# Autodesk Inventor assembly: Placa_base
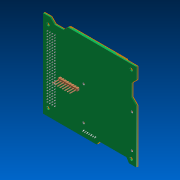
[picture p0: Inventor's stored thumbnail of the model, 180x180]
Saved by Autodesk Inventor 2012 (Build 160160000, 160)
## iProperties
Created: 2015-11-18
Part Number: Placa_base
Document SubType Name: Assembly
Designer: Alex Becerra
Mass: 39.7059 g
Surface Area: 235.798 cm^2
Volume: 15.4172 cm^3
Density: 2.57542 g/cm^3
Author: Alex Becerra
## Documents named in this file (5)
- C:\Users\Thinkpad\Cubesat SUChAI\Mecanica\Modelo_3D\Placa_payloads\Placa_base\Placa_base.iam
- C:\Users\Thinkpad\Cubesat SUChAI\Mecanica\Modelo_3D\Placa_payloads\Placa_base\961108-6804-XX.ipt
- C:\Users\Thinkpad\Cubesat SUChAI\Mecanica\Modelo_3D\Placa_payloads\Placa_base\530140710.ipt
- C:\Users\Thinkpad\Cubesat SUChAI\Mecanica\Modelo_3D\Placa_payloads\Placa_base\pin_header_awl254-dg-g52d.ipt
- C:\Users\Thinkpad\Cubesat SUChAI\Mecanica\Modelo_3D\Placa_payloads\Placa_base\placa_pc104.ipt
## Components (5 placed, 4 different names)
1. 961108-6804-XX:1 — Mate:7, Mate:8, Mate:9
2. 530140710:1 — Mate:10, Mate:11
3. pin_header_awl254-dg-g52d:1 — Mate:1, Mate:3, Mate:4
4. placa_pc104:1 — Mate:1, Mate:2, Mate:3, Mate:4, Mate:5, Mate:6, Mate:7, Mate:8, Mate:9, Mate:10, Mate:11
5. pin_header_awl254-dg-g52d:2 — Mate:2, Mate:5, Mate:6
## Relationships (11: Mate 11)
- Mate:1: pin_header_awl254-dg-g52d:1 ↔ placa_pc104:1
- Mate:2: placa_pc104:1 ↔ pin_header_awl254-dg-g52d:2
- Mate:3: pin_header_awl254-dg-g52d:1 ↔ placa_pc104:1
- Mate:4: pin_header_awl254-dg-g52d:1 ↔ placa_pc104:1
- Mate:5: placa_pc104:1 ↔ pin_header_awl254-dg-g52d:2
- Mate:6: placa_pc104:1 ↔ pin_header_awl254-dg-g52d:2
- Mate:7: 961108-6804-XX:1 ↔ placa_pc104:1
- Mate:8: 961108-6804-XX:1 ↔ placa_pc104:1
- Mate:9: 961108-6804-XX:1 ↔ placa_pc104:1
- Mate:10: 530140710:1 ↔ placa_pc104:1
- Mate:11: 530140710:1 ↔ placa_pc104:1
